# Autodesk Inventor assembly: SoldeerstationAssambly
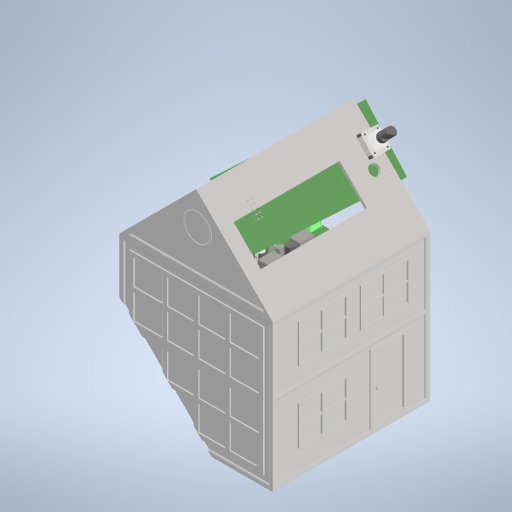
[picture p0: Inventor's stored thumbnail of the model, 512x512]
Saved by Autodesk Inventor 2023 (Build 270158000, 158)
## iProperties
Created: 2023-05-29
Part Number: SoldeerstationAssambly
Document SubType Name: Assembly
Designer: jaspe
Author: jaspe
## Documents named in this file (6)
- C:\Users\jaspe\OneDrive - PXL\Documenten\Electonica-ICT-1e jaar\Project ontwerpen\Ontwerpen\Soldeerstation2\SoldeerstationAssambly.iam
- C:\Users\jaspe\OneDrive - PXL\Documenten\Electonica-ICT-1e jaar\Project ontwerpen\Ontwerpen\Soldeerstation2\HouseSolderingStation.ipt
- C:\Users\jaspe\OneDrive - PXL\Documenten\Electonica-ICT-1e jaar\Project ontwerpen\Ontwerpen\Soldeerstation2\DekselCase.ipt
- C:\Users\jaspe\OneDrive - PXL\Documenten\Electonica-ICT-1e jaar\Project ontwerpen\Ontwerpen\Soldeerstation2\Soldeerstation.iam
- C:\Users\jaspe\OneDrive - PXL\Documenten\Electonica-ICT-1e jaar\Project ontwerpen\Ontwerpen\Soldeerstation2\TraFo.ipt
- C:\Users\jaspe\OneDrive - PXL\Documenten\Electonica-ICT-1e jaar\Project ontwerpen\Ontwerpen\Soldeerstation2\PCB2.iam
## Components (5 placed, 5 different names)
1. HouseSolderingStation:1 — Mate:1, Mate:2, Mate:3, Mate:4, Mate:5
2. DekselCase:1 — Mate:1
3. Soldeerstation:1 [sub-assembly] — Mate:2
4. TraFo:1 — Mate:3
5. PCB2:1 [sub-assembly] — Mate:4, Mate:5
## Relationships (5: Mate 5)
- Mate:1: HouseSolderingStation:1 ↔ DekselCase:1
- Mate:2: HouseSolderingStation:1 ↔ Soldeerstation:1
- Mate:3: HouseSolderingStation:1 ↔ TraFo:1
- Mate:4: HouseSolderingStation:1 ↔ PCB2:1
- Mate:5: HouseSolderingStation:1 ↔ PCB2:1
